# Autodesk Inventor assembly: MainBoard_V1.1
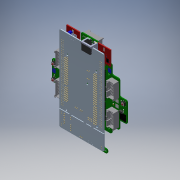
[picture p0: Inventor's stored thumbnail of the model, 180x180]
Saved by Autodesk Inventor 2019 (Build 230136000, 136)
## iProperties
Created: 2019-06-03
Part Number: MainBoard_V1.1
Document SubType Name: Assembly
Designer: jg_ma
Sending System: Autodesk Translation Framework v8.2.0.1029
Preprocessor: ST-DEVELOPER v18
Title: c:\worker\convert-fusion-r04\tmp\job-1\49\output\files\84045320-5f77-4813-9c10-6cf7716fc3ab\677a48ce-5e05-49cf-bbbc-0fea118f8316.stp
## Documents named in this file (13)
- D:\Desktop\Eletronica_Mecanica\MainBoard_V1.1\MainBoard_V1.1.iam
- D:\Desktop\Eletronica_Mecanica\MainBoard_V1.1\PCB Component.iam
- D:\Desktop\Eletronica_Mecanica\MainBoard_V1.1\55917-1010_stp\559171010.ipt
- D:\Desktop\Eletronica_Mecanica\MainBoard_V1.1\55917-2010_stp\559172010.ipt
- D:\Desktop\Eletronica_Mecanica\MainBoard_V1.1\XT60\PDB XT60 PLUG.ipt
- D:\Desktop\Eletronica_Mecanica\MainBoard_V1.1\NRF\nRF24L01-Chip-v13.iam
- D:\Desktop\Eletronica_Mecanica\MainBoard_V1.1\tactile-switches-smd-1.snapshot.7\Tact Switch SMD 4.5x4.5mm.ipt
- D:\Desktop\Eletronica_Mecanica\MainBoard_V1.1\Pinos\2x8.iam
- D:\Desktop\Eletronica_Mecanica\MainBoard_V1.1\Pinos\2x10a.iam
- D:\Desktop\Eletronica_Mecanica\MainBoard_V1.1\Pinos\2x15.iam
- D:\Desktop\Eletronica_Mecanica\MainBoard_V1.1\Pinos\2x17.iam
- D:\Desktop\Eletronica_Mecanica\MainBoard_V1.1\NUCLEO-F429ZI\NUCLEO-F429ZI.iam
- D:\Desktop\Eletronica_Mecanica\MainBoard_V1.1\SlideSwitch\1101M2S3AQE2.ipt
## Components (19 placed, 12 different names)
1. PCB Component:1 [sub-assembly] — Mate:1, Mate:2, Mate:3, Mate:4, Mate:5, Mate:6, Mate:7, Mate:8, Mate:9, Mate:10, Mate:11, Mate:12, Mate:13, Mate:14, Mate:15, Mate:16, Mate:17, Mate:18, Mate:19, Mate:20, Mate:21, Mate:22, Mate:23, Flush:1, Flush:2, Flush:3, Mate:24, Mate:25, Mate:26, Mate:27, Mate:30, Mate:31
2. 559171010:1 — Mate:1, Mate:2
3. 559172010:1 — Mate:3, Mate:7
4. 559172010:2 — Mate:4, Mate:8
5. 559172010:3 — Mate:6, Mate:9
6. 559172010:4 — Mate:5, Mate:10
7. 559172010:5 — Mate:11, Mate:12
8. PDB XT60 PLUG:1 — Mate:13, Mate:14
9. nRF24L01-Chip-v13:1 [sub-assembly] — Mate:15, Mate:16, Mate:17
10. nRF24L01-Chip-v13:2 [sub-assembly] — Mate:18, Mate:19, Mate:20
11. Tact Switch SMD 4.5x4.5mm:1 — Mate:22, Flush:2
12. Tact Switch SMD 4.5x4.5mm:2 — Mate:21, Flush:3
13. Tact Switch SMD 4.5x4.5mm:3 — Mate:23, Flush:1
14. 2x8:1 [sub-assembly] — Mate:24
15. 2x10a:1 [sub-assembly] — Mate:25
16. 2x15:1 [sub-assembly] — Mate:27, Mate:28
17. 2x17:1 [sub-assembly] — Mate:26
18. NUCLEO-F429ZI:1 [sub-assembly] — Mate:28, Mate:30
19. 1101M2S3AQE2:1 — Mate:31
## Relationships (33: Mate 30, Flush 3)
- Mate:1: PCB Component:1 ↔ 559171010:1
- Mate:2: PCB Component:1 ↔ 559171010:1
- Mate:3: PCB Component:1 ↔ 559172010:1
- Mate:4: PCB Component:1 ↔ 559172010:2
- Mate:5: PCB Component:1 ↔ 559172010:4
- Mate:6: PCB Component:1 ↔ 559172010:3
- Mate:7: PCB Component:1 ↔ 559172010:1
- Mate:8: PCB Component:1 ↔ 559172010:2
- Mate:9: PCB Component:1 ↔ 559172010:3
- Mate:10: PCB Component:1 ↔ 559172010:4
- Mate:11: PCB Component:1 ↔ 559172010:5
- Mate:12: PCB Component:1 ↔ 559172010:5
- Mate:13: PCB Component:1 ↔ PDB XT60 PLUG:1
- Mate:14: PCB Component:1 ↔ PDB XT60 PLUG:1
- Mate:15: PCB Component:1 ↔ nRF24L01-Chip-v13:1
- Mate:16: PCB Component:1 ↔ nRF24L01-Chip-v13:1
- Mate:17: PCB Component:1 ↔ nRF24L01-Chip-v13:1
- Mate:18: PCB Component:1 ↔ nRF24L01-Chip-v13:2
- Mate:19: PCB Component:1 ↔ nRF24L01-Chip-v13:2
- Mate:20: PCB Component:1 ↔ nRF24L01-Chip-v13:2
- Mate:21: PCB Component:1 ↔ Tact Switch SMD 4.5x4.5mm:2
- Mate:22: PCB Component:1 ↔ Tact Switch SMD 4.5x4.5mm:1
- Mate:23: PCB Component:1 ↔ Tact Switch SMD 4.5x4.5mm:3
- Flush:1 (1.8 mm): PCB Component:1 ↔ Tact Switch SMD 4.5x4.5mm:3
- Flush:2 (1.8 mm): PCB Component:1 ↔ Tact Switch SMD 4.5x4.5mm:1
- Flush:3 (1.8 mm): PCB Component:1 ↔ Tact Switch SMD 4.5x4.5mm:2
- Mate:24: PCB Component:1 ↔ 2x8:1
- Mate:25: PCB Component:1 ↔ 2x10a:1
- Mate:26: PCB Component:1 ↔ 2x17:1
- Mate:27: PCB Component:1 ↔ 2x15:1
- Mate:28 (0.04 mm): 2x15:1 ↔ NUCLEO-F429ZI:1
- Mate:30: PCB Component:1 ↔ NUCLEO-F429ZI:1
- Mate:31: PCB Component:1 ↔ 1101M2S3AQE2:1
